# Autodesk Inventor assembly: Intake Pivot Assembly
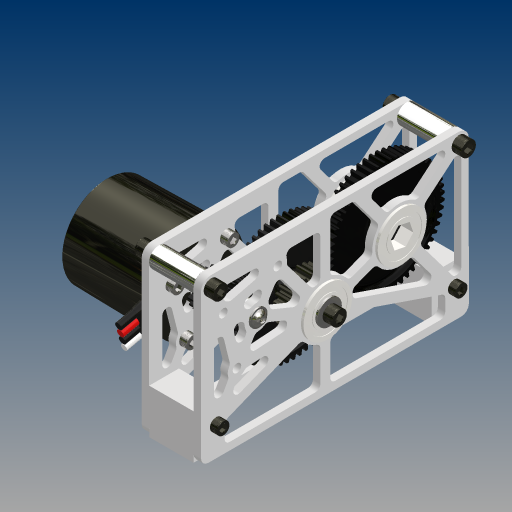
[picture p0: Inventor's stored thumbnail of the model, 512x512]
Saved by Autodesk Inventor 2024.3 (Build 283343000, 343)
## iProperties
Created: 2024-08-01
Part Number: Intake Pivot Assembly
Document SubType Name: Assembly
Designer: Kenji
Author: Kenji
## Documents named in this file (19)
- C:\Users\Kenji\Documents\GitHub\1622-2024-Summer-CAD-A-Thon\Intake\Intake Pivot Assembly.iam
- C:\Users\Kenji\Documents\GitHub\1622-2024-Summer-CAD-A-Thon\Intake\Intake Pivot Gearbox.ipt
- C:\Users\Kenji\Documents\GitHub\1622-2024-Summer-CAD-A-Thon\COTS Library\Motors\COTS_REV-21-1650-V1.1_Neo1.1.ipt
- C:\Users\Kenji\Documents\GitHub\1622-2024-Summer-CAD-A-Thon\Intake\WCP-1236 (1).ipt
- C:\Users\Kenji\Documents\GitHub\1622-2024-Summer-CAD-A-Thon\Intake\WCP-0186.ipt
- C:\Users\Kenji\Documents\GitHub\1622-2024-Summer-CAD-A-Thon\COTS Library\Motion\Bearings\COTS_WCP-0783_1.125ODHexBearing.ipt
- C:\Users\Kenji\Documents\GitHub\1622-2024-Summer-CAD-A-Thon\COTS Library\Fasteners\Bolts\Socket-Head\10-32\COTS_91251A340__3-18in long_Black-Oxide Alloy Steel Socket Head.ipt
- C:\Users\Kenji\Documents\GitHub\1622-2024-Summer-CAD-A-Thon\Intake\Intake Pivot Spacer 1.ipt
- C:\Users\Kenji\Documents\GitHub\1622-2024-Summer-CAD-A-Thon\Intake\Intake Pivot Spacer 2.ipt
- C:\Users\Kenji\Documents\GitHub\1622-2024-Summer-CAD-A-Thon\Intake\Intake Pivot Hex Shaft.ipt
- C:\Users\Kenji\Documents\GitHub\1622-2024-Summer-CAD-A-Thon\Intake\Intake Pivot Spacer 3.ipt
- C:\Users\Kenji\Documents\GitHub\1622-2024-Summer-CAD-A-Thon\COTS Library\Fasteners\Bolts\Socket-Head\0.25-20\COTS_91251A537_Black-Oxide Alloy Steel Socket Head Screw.ipt
- C:\Users\Kenji\Documents\GitHub\1622-2024-Summer-CAD-A-Thon\COTS Library\Fasteners\Washers\COTS_90107A029_316 Stainless Steel Washer.ipt
- C:\Users\Kenji\Documents\GitHub\1622-2024-Summer-CAD-A-Thon\COTS Library\Fasteners\Washers\COTS_91860A047_Size10Washer.ipt
- C:\Users\Kenji\Documents\GitHub\1622-2024-Summer-CAD-A-Thon\COTS Library\Fasteners\Bolts\Button-Head\10-32\COTS_92949A265_1-2in long Stainless Steel Button Head Screw.ipt
- C:\Users\Kenji\Documents\GitHub\1622-2024-Summer-CAD-A-Thon\COTS Library\Motion\Gears\20DP gears\Steel\0.5in hex\COTS_WCP-0736_Steel_24T20DPGear.ipt
- C:\Users\Kenji\Documents\GitHub\1622-2024-Summer-CAD-A-Thon\Intake\WCP-0185.ipt
- C:\Users\Kenji\Documents\GitHub\1622-2024-Summer-CAD-A-Thon\Intake\Intake Pivot Billet.ipt
- C:\Users\Kenji\Documents\GitHub\1622-2024-Summer-CAD-A-Thon\COTS Library\Fasteners\Bolts\Socket-Head\10-32\COTS_91251A342_1-2in Long_Black-Oxide Alloy Steel Socket Head.ipt
## Components (35 placed, 18 different names)
1. Intake Pivot Gearbox:1 — Mate:1, Mate:2, Mate:17, Mate:18, Mate:19, Mate:20, Mate:42, Mate:44, Mate:45, Mate:48, Mate:49, Mate:52, Mate:64, Mate:73, Flush:4, Mate:76, Flush:5, Mate:77, Mate:80, Mate:81, Mate:83
2. Intake Pivot Gearbox:2 — Mate:1, Mate:2, Mate:3, Mate:5, Mate:7, Mate:8, Mate:9, Mate:10, Mate:11, Mate:12, Mate:24, Mate:27, Mate:28, Mate:30, Mate:31, Mate:39, Mate:40, Mate:41, Mate:43, Mate:46, Mate:47, Mate:50, Mate:51, Mate:67, Mate:74, Mate:75, Mate:78, Mate:79, Mate:82, Mate:84
3. COTS_REV-21-1650-V1.1_Neo1.1:1 — Mate:3, Mate:5, Mate:6, Mate:33, Mate:39, Mate:63
4. WCP-1236 (1):1 — Mate:6, Mate:7, Mate:34
5. WCP-0186:1 — Mate:8, Mate:13, Mate:68
6. COTS_WCP-0783_1.125ODHexBearing:1 — Mate:17, Mate:20, Mate:38, Flush:3, Mate:56, Mate:69
7. COTS_WCP-0783_1.125ODHexBearing:2 — Mate:18, Mate:19
8. COTS_WCP-0783_1.125ODHexBearing:3 — Mate:9, Mate:10, Mate:13, Mate:60
9. COTS_WCP-0783_1.125ODHexBearing:4 — Mate:11, Mate:12, Mate:35, Mate:72
10. COTS_91251A340__3-18in long_Black-Oxide Alloy Steel Socket Head:2 — Mate:24, Mate:30
11. COTS_91251A340__3-18in long_Black-Oxide Alloy Steel Socket Head:4 — Mate:31, Mate:40
12. COTS_91251A340__3-18in long_Black-Oxide Alloy Steel Socket Head:6 — Mate:27, Mate:28
13. Intake Pivot Spacer 1:1 — Mate:33, Mate:34
14. Intake Pivot Spacer 2:1 — Mate:35, Mate:70, Mate:71, Mate:72
15. Intake Pivot Hex Shaft:2 — Mate:38, Flush:3, Mate:55, Mate:59
16. Intake Pivot Spacer 3:1 — Mate:41, Mate:42
17. Intake Pivot Spacer 3:2 — Mate:43, Mate:44, Mate:67
18. COTS_91251A537_Black-Oxide Alloy Steel Socket Head Screw:1 — Mate:45, Mate:48
19. COTS_91251A537_Black-Oxide Alloy Steel Socket Head Screw:2 — Mate:46, Mate:47
20. COTS_91251A537_Black-Oxide Alloy Steel Socket Head Screw:3 — Mate:49, Mate:52
21. COTS_91251A537_Black-Oxide Alloy Steel Socket Head Screw:4 — Mate:50, Mate:51
22. COTS_91251A537_Black-Oxide Alloy Steel Socket Head Screw:6 — Mate:53, Mate:54, Mate:55
23. COTS_91251A537_Black-Oxide Alloy Steel Socket Head Screw:7 — Mate:57, Mate:58, Mate:59
24. COTS_90107A029_316 Stainless Steel Washer:1 — Mate:53, Mate:54, Mate:56
25. COTS_90107A029_316 Stainless Steel Washer:2 — Mate:57, Mate:58, Mate:60
26. COTS_91860A047_Size10Washer:1 — Mate:61, Mate:62, Mate:63, Mate:64
27. COTS_92949A265_1-2in long Stainless Steel Button Head Screw:1 — Mate:61, Mate:62
28. COTS_WCP-0736_Steel_24T20DPGear:1 — Mate:68, Mate:69
29. WCP-0185:1 — Mate:70, Mate:71
30. Intake Pivot Billet:1 — Mate:75, Mate:76, Flush:5
31. Intake Pivot Billet:2 — Mate:73, Mate:74, Flush:4
32. COTS_91251A342_1-2in Long_Black-Oxide Alloy Steel Socket Head:1 — Mate:77, Mate:80
33. COTS_91251A342_1-2in Long_Black-Oxide Alloy Steel Socket Head:2 — Mate:78, Mate:79
34. COTS_91251A342_1-2in Long_Black-Oxide Alloy Steel Socket Head:3 — Mate:81, Mate:83
35. COTS_91251A342_1-2in Long_Black-Oxide Alloy Steel Socket Head:4 — Mate:82, Mate:84
## Relationships (72: Mate 69, Flush 3)
- Mate:1: Intake Pivot Gearbox:1 ↔ Intake Pivot Gearbox:2
- Mate:2: Intake Pivot Gearbox:1 ↔ Intake Pivot Gearbox:2
- Mate:3: Intake Pivot Gearbox:2 ↔ COTS_REV-21-1650-V1.1_Neo1.1:1
- Mate:5: Intake Pivot Gearbox:2 ↔ COTS_REV-21-1650-V1.1_Neo1.1:1
- Mate:6: COTS_REV-21-1650-V1.1_Neo1.1:1 ↔ WCP-1236 (1):1
- Mate:7: Intake Pivot Gearbox:2 ↔ WCP-1236 (1):1
- Mate:8: Intake Pivot Gearbox:2 ↔ WCP-0186:1
- Mate:9: Intake Pivot Gearbox:2 ↔ COTS_WCP-0783_1.125ODHexBearing:3
- Mate:10: Intake Pivot Gearbox:2 ↔ COTS_WCP-0783_1.125ODHexBearing:3
- Mate:11: Intake Pivot Gearbox:2 ↔ COTS_WCP-0783_1.125ODHexBearing:4
- Mate:12: Intake Pivot Gearbox:2 ↔ COTS_WCP-0783_1.125ODHexBearing:4
- Mate:13: WCP-0186:1 ↔ COTS_WCP-0783_1.125ODHexBearing:3
- Mate:17: Intake Pivot Gearbox:1 ↔ COTS_WCP-0783_1.125ODHexBearing:1
- Mate:18: Intake Pivot Gearbox:1 ↔ COTS_WCP-0783_1.125ODHexBearing:2
- Mate:19: Intake Pivot Gearbox:1 ↔ COTS_WCP-0783_1.125ODHexBearing:2
- Mate:20: Intake Pivot Gearbox:1 ↔ COTS_WCP-0783_1.125ODHexBearing:1
- Mate:24: Intake Pivot Gearbox:2 ↔ COTS_91251A340__3-18in long_Black-Oxide Alloy Steel Socket Head:2
- Mate:27: Intake Pivot Gearbox:2 ↔ COTS_91251A340__3-18in long_Black-Oxide Alloy Steel Socket Head:6
- Mate:28: Intake Pivot Gearbox:2 ↔ COTS_91251A340__3-18in long_Black-Oxide Alloy Steel Socket Head:6
- Mate:30: Intake Pivot Gearbox:2 ↔ COTS_91251A340__3-18in long_Black-Oxide Alloy Steel Socket Head:2
- Mate:31: Intake Pivot Gearbox:2 ↔ COTS_91251A340__3-18in long_Black-Oxide Alloy Steel Socket Head:4
- Mate:33: COTS_REV-21-1650-V1.1_Neo1.1:1 ↔ Intake Pivot Spacer 1:1
- Mate:34: WCP-1236 (1):1 ↔ Intake Pivot Spacer 1:1
- Mate:35: COTS_WCP-0783_1.125ODHexBearing:4 ↔ Intake Pivot Spacer 2:1
- Mate:38: COTS_WCP-0783_1.125ODHexBearing:1 ↔ Intake Pivot Hex Shaft:2
- Flush:3: COTS_WCP-0783_1.125ODHexBearing:1 ↔ Intake Pivot Hex Shaft:2
- Mate:39: Intake Pivot Gearbox:2 ↔ COTS_REV-21-1650-V1.1_Neo1.1:1
- Mate:40: Intake Pivot Gearbox:2 ↔ COTS_91251A340__3-18in long_Black-Oxide Alloy Steel Socket Head:4
- Mate:41: Intake Pivot Gearbox:2 ↔ Intake Pivot Spacer 3:1
- Mate:42: Intake Pivot Gearbox:1 ↔ Intake Pivot Spacer 3:1
- Mate:43: Intake Pivot Gearbox:2 ↔ Intake Pivot Spacer 3:2
- Mate:44: Intake Pivot Gearbox:1 ↔ Intake Pivot Spacer 3:2
- Mate:45: Intake Pivot Gearbox:1 ↔ COTS_91251A537_Black-Oxide Alloy Steel Socket Head Screw:1
- Mate:46: Intake Pivot Gearbox:2 ↔ COTS_91251A537_Black-Oxide Alloy Steel Socket Head Screw:2
- Mate:47: Intake Pivot Gearbox:2 ↔ COTS_91251A537_Black-Oxide Alloy Steel Socket Head Screw:2
- Mate:48: Intake Pivot Gearbox:1 ↔ COTS_91251A537_Black-Oxide Alloy Steel Socket Head Screw:1
- Mate:49: Intake Pivot Gearbox:1 ↔ COTS_91251A537_Black-Oxide Alloy Steel Socket Head Screw:3
- Mate:50: Intake Pivot Gearbox:2 ↔ COTS_91251A537_Black-Oxide Alloy Steel Socket Head Screw:4
- Mate:51: Intake Pivot Gearbox:2 ↔ COTS_91251A537_Black-Oxide Alloy Steel Socket Head Screw:4
- Mate:52: Intake Pivot Gearbox:1 ↔ COTS_91251A537_Black-Oxide Alloy Steel Socket Head Screw:3
- Mate:53: COTS_91251A537_Black-Oxide Alloy Steel Socket Head Screw:6 ↔ COTS_90107A029_316 Stainless Steel Washer:1
- Mate:54: COTS_91251A537_Black-Oxide Alloy Steel Socket Head Screw:6 ↔ COTS_90107A029_316 Stainless Steel Washer:1
- Mate:55: Intake Pivot Hex Shaft:2 ↔ COTS_91251A537_Black-Oxide Alloy Steel Socket Head Screw:6
- Mate:56: COTS_WCP-0783_1.125ODHexBearing:1 ↔ COTS_90107A029_316 Stainless Steel Washer:1
- Mate:57: COTS_91251A537_Black-Oxide Alloy Steel Socket Head Screw:7 ↔ COTS_90107A029_316 Stainless Steel Washer:2
- Mate:58: COTS_91251A537_Black-Oxide Alloy Steel Socket Head Screw:7 ↔ COTS_90107A029_316 Stainless Steel Washer:2
- Mate:59: Intake Pivot Hex Shaft:2 ↔ COTS_91251A537_Black-Oxide Alloy Steel Socket Head Screw:7
- Mate:60: COTS_WCP-0783_1.125ODHexBearing:3 ↔ COTS_90107A029_316 Stainless Steel Washer:2
- Mate:61: COTS_91860A047_Size10Washer:1 ↔ COTS_92949A265_1-2in long Stainless Steel Button Head Screw:1
- Mate:62: COTS_91860A047_Size10Washer:1 ↔ COTS_92949A265_1-2in long Stainless Steel Button Head Screw:1
- Mate:63: COTS_REV-21-1650-V1.1_Neo1.1:1 ↔ COTS_91860A047_Size10Washer:1
- Mate:64: Intake Pivot Gearbox:1 ↔ COTS_91860A047_Size10Washer:1
- Mate:67: Intake Pivot Gearbox:2 ↔ Intake Pivot Spacer 3:2
- Mate:68: WCP-0186:1 ↔ COTS_WCP-0736_Steel_24T20DPGear:1
- Mate:69: COTS_WCP-0783_1.125ODHexBearing:1 ↔ COTS_WCP-0736_Steel_24T20DPGear:1
- Mate:70: Intake Pivot Spacer 2:1 ↔ WCP-0185:1
- Mate:71: Intake Pivot Spacer 2:1 ↔ WCP-0185:1
- Mate:72: COTS_WCP-0783_1.125ODHexBearing:4 ↔ Intake Pivot Spacer 2:1
- Mate:73: Intake Pivot Gearbox:1 ↔ Intake Pivot Billet:2
- Mate:74: Intake Pivot Gearbox:2 ↔ Intake Pivot Billet:2
- Flush:4: Intake Pivot Gearbox:1 ↔ Intake Pivot Billet:2
- Mate:75: Intake Pivot Gearbox:2 ↔ Intake Pivot Billet:1
- Mate:76: Intake Pivot Gearbox:1 ↔ Intake Pivot Billet:1
- Flush:5: Intake Pivot Gearbox:1 ↔ Intake Pivot Billet:1
- Mate:77: Intake Pivot Gearbox:1 ↔ COTS_91251A342_1-2in Long_Black-Oxide Alloy Steel Socket Head:1
- Mate:78: Intake Pivot Gearbox:2 ↔ COTS_91251A342_1-2in Long_Black-Oxide Alloy Steel Socket Head:2
- Mate:79: Intake Pivot Gearbox:2 ↔ COTS_91251A342_1-2in Long_Black-Oxide Alloy Steel Socket Head:2
- Mate:80: Intake Pivot Gearbox:1 ↔ COTS_91251A342_1-2in Long_Black-Oxide Alloy Steel Socket Head:1
- Mate:81: Intake Pivot Gearbox:1 ↔ COTS_91251A342_1-2in Long_Black-Oxide Alloy Steel Socket Head:3
- Mate:82: Intake Pivot Gearbox:2 ↔ COTS_91251A342_1-2in Long_Black-Oxide Alloy Steel Socket Head:4
- Mate:83: Intake Pivot Gearbox:1 ↔ COTS_91251A342_1-2in Long_Black-Oxide Alloy Steel Socket Head:3
- Mate:84: Intake Pivot Gearbox:2 ↔ COTS_91251A342_1-2in Long_Black-Oxide Alloy Steel Socket Head:4
